# Autodesk Inventor assembly: 45 Degree Hinge with Wood Screws And Cup Fixing Wood Screws
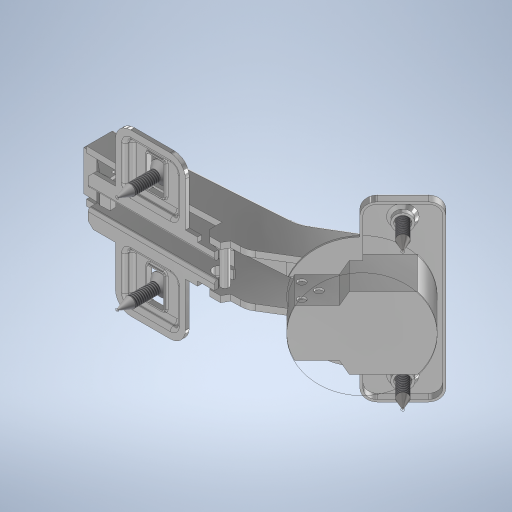
[picture p0: Inventor's stored thumbnail of the model, 512x512]
Saved by Autodesk Inventor 2024 (Build 280153000, 153)
## iProperties
Created: 2014-03-31
Part Number: 45 Degree Hinge with Wood Screws And Cup Fixing Wood Screws
Document SubType Name: Assembly
Designer: G. Kazokaitis
Author: G. Kazokaitis
## Documents named in this file (8)
- C:\W4INV 2024 Design\_LIBRARY\Hinges\45 DEGREE HINGE\45 Degree Hinge with Wood Screws And Cup Fixing Wood Screws.iam
- C:\W4INV 2024 Design\LIBRARY\Hinges\Parts\45 Degree hinge\Lever.ipt
- C:\W4INV 2024 Design\LIBRARY\Hinges\Parts\45 Degree hinge\Linkage.ipt
- C:\W4INV 2024 Design\LIBRARY\Hinges\45 DEGREE HINGE.iam
- C:\W4INV 2024 Design\_LIBRARY\Hinges\Parts\45 Degree hinge\Case and plate\45 degree Hinge with Wood Screw.ipt
- C:\W4INV 2024 Design\_LIBRARY\Hinges\Parts\45 Degree hinge\Cup for hinge\Cup for hinge with wood screws.ipt
- C:\W4INV 2023 Design\LIBRARY\Hinges\Parts\45 Degree hinge\Case and plate.ipt
- C:\W4INV 2023 Design\LIBRARY\Hinges\Parts\45 Degree hinge\Cup for hinge.ipt
## Components (4 placed, 4 different names)
1. 45 degree Hinge with Wood Screw:1 — Mate:1, Angle:1, Flush:1, Mate:3, Flush:2, Mate:4, Mate:5, Drive angle, Flush:3
2. Lever:1 — Mate:4, Mate:5, Mate:7, Mate:8
3. Linkage:1 — Mate:3, Flush:2, Mate:6
4. Cup for hinge with wood screws:1 — Mate:6, Mate:7, Mate:8, Drive angle
## Relationships (12: Mate 7, Flush 3, Angle 2)
- Mate:1: 45 degree Hinge with Wood Screw:1
- Angle:1 (0 deg): 45 degree Hinge with Wood Screw:1
- Flush:1 (8.575 mm): 45 degree Hinge with Wood Screw:1
- Mate:3: 45 degree Hinge with Wood Screw:1 ↔ Linkage:1
- Flush:2 (1.125 mm): 45 degree Hinge with Wood Screw:1 ↔ Linkage:1
- Mate:4: 45 degree Hinge with Wood Screw:1 ↔ Lever:1
- Mate:5 (1.3 mm): 45 degree Hinge with Wood Screw:1 ↔ Lever:1
- Mate:6: Linkage:1 ↔ Cup for hinge with wood screws:1
- Mate:7: Lever:1 ↔ Cup for hinge with wood screws:1
- Mate:8 (3.275 mm): Lever:1 ↔ Cup for hinge with wood screws:1
- Drive angle [Angle] (135 deg): 45 degree Hinge with Wood Screw:1 ↔ Cup for hinge with wood screws:1
- Flush:3 (-2.75 mm): 45 degree Hinge with Wood Screw:1
